# Autodesk Inventor assembly: Time
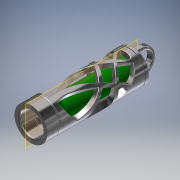
[picture p0: Inventor's stored thumbnail of the model, 180x180]
Saved by Autodesk Inventor 2019 (Build 230136000, 136)
## iProperties
Created: 2019-05-03
Part Number: Time
Document SubType Name: Assembly
Designer: Jorian Brusind
Author: Jorian Brusind
## Documents named in this file (3)
- C:\Users\Jorian Brusind\Documents\GitHub\PersonalProjects\Inventor Projects\Infinity\Time.iam
- C:\Users\Jorian Brusind\Documents\GitHub\PersonalProjects\Inventor Projects\Infinity\Green.ipt
- C:\Users\Jorian Brusind\Documents\GitHub\PersonalProjects\Inventor Projects\Infinity\Agamoto.ipt
## Components (2 placed, 2 different names)
1. Green:1 — Mate:1, Mate:2
2. Agamoto:1 — Mate:1, Mate:2
## Relationships (2: Mate 2)
- Mate:1: Green:1 ↔ Agamoto:1
- Mate:2: Green:1 ↔ Agamoto:1
